# Autodesk Inventor assembly: GRIPPER_ASSEM_FINAL
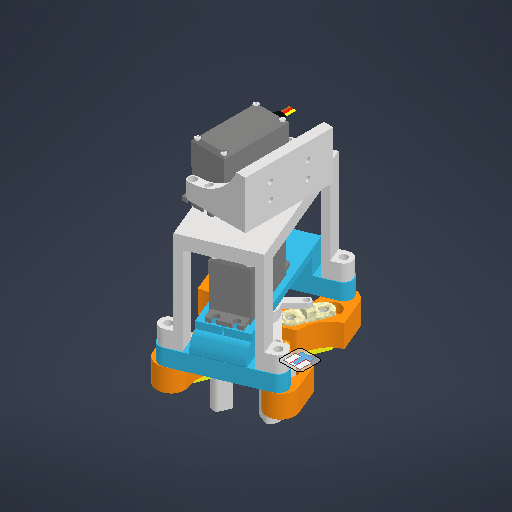
[picture p0: Inventor's stored thumbnail of the model, 512x512]
Saved by Autodesk Inventor 2025.1 (Build 291241000, 241)
## iProperties
Created: 2024-11-11
Part Number: GRIPPER_ASSEM_FINAL
Document SubType Name: Assembly
Designer: m_kni
Author: m_kni
## Documents named in this file (11)
- C:\Users\jerem\Documents\GitHub\Perovskite-Automated-Synthesis-System\CAD\Gripper\GRIPPER_ASSEM_FINAL.iam
- C:\Users\jerem\Documents\GitHub\Perovskite-Automated-Synthesis-System\CAD\Gripper\SERVO_TO_TOOLHEAD.ipt
- C:\Users\jerem\Documents\GitHub\Perovskite-Automated-Synthesis-System\CAD\Non 3D Printed Parts\Motors and Servos\Servo MG996R.ipt
- C:\Users\jerem\Documents\GitHub\Perovskite-Automated-Synthesis-System\CAD\Gripper\ATTACHMENT_TOOLHEAD_GRIPPER.ipt
- C:\Users\jerem\Documents\GitHub\Perovskite-Automated-Synthesis-System\CAD\Gripper\SERVO_MOUNT_TOBASE.ipt
- C:\Users\jerem\Documents\GitHub\Perovskite-Automated-Synthesis-System\CAD\Gripper\BaseSketchGrabberrev2.0.ipt
- C:\Users\jerem\Documents\GitHub\Perovskite-Automated-Synthesis-System\CAD\Gripper\5x5x11bearing.ipt
- C:\Users\jerem\Documents\GitHub\Perovskite-Automated-Synthesis-System\CAD\Gripper\spinner.ipt
- C:\Users\jerem\Documents\GitHub\Perovskite-Automated-Synthesis-System\CAD\Gripper\bearing plate.ipt
- C:\Users\jerem\Documents\GitHub\Perovskite-Automated-Synthesis-System\CAD\Gripper\arm.ipt
- C:\Users\jerem\Documents\GitHub\Perovskite-Automated-Synthesis-System\CAD\Gripper\LINKV2.ipt
## Components (32 placed, 10 different names)
1. SERVO_TO_TOOLHEAD:1 — Insert:1, Insert:2
2. Servo MG996R:1 — Insert:1, Insert:2, Insert:3
3. ATTACHMENT_TOOLHEAD_GRIPPER:1 — Insert:3, Insert:4, Angle:1, Angle:2
4. SERVO_MOUNT_TOBASE:1 — Insert:4, Angle:1, Insert:5, Insert:28, Insert:29
5. BaseSketchGrabberrev2.0:1 — Insert:5, Angle:2, Insert:6, Insert:8, Insert:9, Insert:10, Insert:11, Insert:12, Insert:13, Insert:14, Insert:15, Angle:3, Angle:4, Angle:5, Angle:6, Angle:7, Angle:8, Angle:9, Angle:10
6. 5x5x11bearing:1 — Insert:6, Insert:7
7. 5x5x11bearing:2 — Insert:15, Insert:25
8. 5x5x11bearing:3 — Insert:14, Insert:26
9. 5x5x11bearing:4 — Insert:13, Insert:24
10. 5x5x11bearing:5 — Insert:11, Insert:17
11. 5x5x11bearing:6 — Insert:12, Insert:27
12. 5x5x11bearing:7 — Insert:9, Insert:21
13. 5x5x11bearing:8 — Insert:8, Insert:20
14. 5x5x11bearing:9 — Insert:10, Insert:16
15. spinner:1 — Insert:7
16. bearing plate:1 — Insert:17, Angle:4, Insert:18, Insert:31
17. bearing plate:2 — Insert:16, Angle:3, Insert:19, Insert:30
18. bearing plate:3 — Insert:20, Angle:5, Insert:23, Insert:33
19. bearing plate:4 — Insert:21, Angle:6, Insert:22, Insert:32
20. 5x5x11bearing:10 — Insert:19
21. 5x5x11bearing:11 — Insert:22
22. 5x5x11bearing:12 — Insert:23
23. 5x5x11bearing:14 — Insert:18
24. arm:1 — Insert:24, Angle:7
25. arm:2 — Insert:25, Angle:8
26. arm:3 — Insert:26, Angle:9
27. arm:4 — Insert:27, Angle:10
28. Servo MG996R:2 — Insert:28, Insert:29
29. LINKV2:1 — Insert:30
30. LINKV2:2 — Insert:31
31. LINKV2:3 — Insert:32
32. LINKV2:4 — Insert:33
## Relationships (43: Insert 33, Angle 10)
- Insert:1: SERVO_TO_TOOLHEAD:1 ↔ Servo MG996R:1
- Insert:2: SERVO_TO_TOOLHEAD:1 ↔ Servo MG996R:1
- Insert:3 (1.27 mm): Servo MG996R:1 ↔ ATTACHMENT_TOOLHEAD_GRIPPER:1
- Insert:4: ATTACHMENT_TOOLHEAD_GRIPPER:1 ↔ SERVO_MOUNT_TOBASE:1
- Angle:1 (0 deg): ATTACHMENT_TOOLHEAD_GRIPPER:1 ↔ SERVO_MOUNT_TOBASE:1
- Insert:5: SERVO_MOUNT_TOBASE:1 ↔ BaseSketchGrabberrev2.0:1
- Angle:2 (0 deg): ATTACHMENT_TOOLHEAD_GRIPPER:1 ↔ BaseSketchGrabberrev2.0:1
- Insert:6: BaseSketchGrabberrev2.0:1 ↔ 5x5x11bearing:1
- Insert:7 (0.508 mm): 5x5x11bearing:1 ↔ spinner:1
- Insert:8: BaseSketchGrabberrev2.0:1 ↔ 5x5x11bearing:8
- Insert:9: BaseSketchGrabberrev2.0:1 ↔ 5x5x11bearing:7
- Insert:10: BaseSketchGrabberrev2.0:1 ↔ 5x5x11bearing:9
- Insert:11: BaseSketchGrabberrev2.0:1 ↔ 5x5x11bearing:5
- Insert:12: BaseSketchGrabberrev2.0:1 ↔ 5x5x11bearing:6
- Insert:13: BaseSketchGrabberrev2.0:1 ↔ 5x5x11bearing:4
- Insert:14: BaseSketchGrabberrev2.0:1 ↔ 5x5x11bearing:3
- Insert:15: BaseSketchGrabberrev2.0:1 ↔ 5x5x11bearing:2
- Insert:16: 5x5x11bearing:9 ↔ bearing plate:2
- Angle:3 (0 deg): BaseSketchGrabberrev2.0:1 ↔ bearing plate:2
- Insert:17: 5x5x11bearing:5 ↔ bearing plate:1
- Angle:4 (0 deg): BaseSketchGrabberrev2.0:1 ↔ bearing plate:1
- Insert:18: bearing plate:1 ↔ 5x5x11bearing:14
- Insert:19: bearing plate:2 ↔ 5x5x11bearing:10
- Insert:20: 5x5x11bearing:8 ↔ bearing plate:3
- Angle:5 (0 deg): BaseSketchGrabberrev2.0:1 ↔ bearing plate:3
- Insert:21: 5x5x11bearing:7 ↔ bearing plate:4
- Angle:6 (180 deg): BaseSketchGrabberrev2.0:1 ↔ bearing plate:4
- Insert:22: bearing plate:4 ↔ 5x5x11bearing:11
- Insert:23: bearing plate:3 ↔ 5x5x11bearing:12
- Insert:24: 5x5x11bearing:4 ↔ arm:1
- Angle:7 (0 deg): BaseSketchGrabberrev2.0:1 ↔ arm:1
- Insert:25: 5x5x11bearing:2 ↔ arm:2
- Angle:8 (0 deg): BaseSketchGrabberrev2.0:1 ↔ arm:2
- Insert:26: 5x5x11bearing:3 ↔ arm:3
- Angle:9 (0 deg): BaseSketchGrabberrev2.0:1 ↔ arm:3
- Insert:27: 5x5x11bearing:6 ↔ arm:4
- Angle:10 (0 deg): BaseSketchGrabberrev2.0:1 ↔ arm:4
- Insert:28: SERVO_MOUNT_TOBASE:1 ↔ Servo MG996R:2
- Insert:29: SERVO_MOUNT_TOBASE:1 ↔ Servo MG996R:2
- Insert:30: bearing plate:2 ↔ LINKV2:1
- Insert:31: bearing plate:1 ↔ LINKV2:2
- Insert:32: bearing plate:4 ↔ LINKV2:3
- Insert:33: bearing plate:3 ↔ LINKV2:4
## Named parameters: Finish1_Area = 165.947, Finish1_Thickness = 0.05 mm
note: some values were not read from the file. Shown as the stored number, unit unknown: "Finish1_Area".
